# Autodesk Inventor assembly: cloudcase
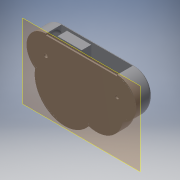
[picture p0: Inventor's stored thumbnail of the model, 180x180]
Saved by Autodesk Inventor 2018.1 (Build 221171000, 171)
## iProperties
Created: 2018-06-29
Part Number: cloudcase
Document SubType Name: Assembly
Designer: erwin
Author: erwin
## Documents named in this file (4)
- C:\Users\erwin\Documents\GitHub\cloudberry-case\design\new\cloudcase.iam
- C:\Users\erwin\Documents\GitHub\cloudberry-case\design\new\board.ipt
- C:\Users\erwin\Documents\GitHub\cloudberry-case\design\new\bottom.ipt
- C:\Users\erwin\Documents\GitHub\cloudberry-case\design\new\cap.ipt
## Components (3 placed, 3 different names)
1. board:1 — Flush:1, Flush:2
2. bottom:1 — Flush:1, Flush:2, Flush:3, Flush:4
3. cap:1 — Flush:3, Flush:4
## Relationships (4: Flush 4)
- Flush:1: board:1 ↔ bottom:1
- Flush:2 (3 mm): board:1 ↔ bottom:1
- Flush:3: bottom:1 ↔ cap:1
- Flush:4: bottom:1 ↔ cap:1
